# Autodesk Inventor assembly: mini sand
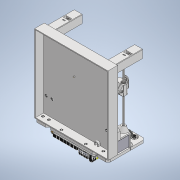
[picture p0: Inventor's stored thumbnail of the model, 180x180]
Saved by Autodesk Inventor 2022 (Build 260153000, 153)
## iProperties
Created: 2022-04-23
Part Number: mini sand
Document SubType Name: Assembly
Designer: Administrator
Title: mini sand v11
Author: Administrator
## Documents named in this file (29)
- Y:\Projects\Mini_Sand_Table\Mini Sand Table.iam
- Y:\Projects\Mini_Sand_Table\4mm x 140mm Rod.ipt
- Y:\Projects\Mini_Sand_Table\603ZZ Roller Bearing.ipt
- Y:\Projects\Mini_Sand_Table\4mm x 130mm Rod.ipt
- Y:\Projects\Mini_Sand_Table\GT2 16T Pulley.ipt
- Y:\Projects\Mini_Sand_Table\magnet.ipt
- Y:\Projects\Mini_Sand_Table\LM4UU.ipt
- Y:\Projects\Mini_Sand_Table\Table Top.ipt
- Y:\Projects\Mini_Sand_Table\NEMA 11.ipt
- Y:\Projects\Mini_Sand_Table\Belt Retainer.ipt
- Y:\Projects\Mini_Sand_Table\Magnet Mount Lower.ipt
- Y:\Projects\Mini_Sand_Table\XY Joiner HSI.iam
- Y:\Projects\Mini_Sand_Table\Idle Bearing Mount HSI.iam
- Y:\Projects\Mini_Sand_Table\M3 Hex Nut.ipt
- Y:\Projects\Mini_Sand_Table\Ball.ipt
- Y:\Projects\Mini_Sand_Table\SKR Mini E3 v3.0.ipt
- Y:\Projects\Mini_Sand_Table\Sand Cover.ipt
- Y:\Projects\Mini_Sand_Table\Magnet Mount HSI.iam
- Y:\Projects\Mini_Sand_Table\Motor Mount HSI.iam
- Y:\Projects\Mini_Sand_Table\Driver Board Mount HSI.iam
- Y:\Projects\Mini_Sand_Table\M3 x 4 mm SHCS.ipt
- Y:\Projects\Mini_Sand_Table\M3 x 25 mm  SHCS.ipt
- Y:\Projects\Mini_Sand_Table\M2.5 x 10 mm SHCS.ipt
- Y:\Projects\Mini_Sand_Table\M2.5 x 6 mm SHCS.ipt
- Y:\Projects\Mini_Sand_Table\M3 x 16 mm FHCS.ipt
- Y:\Projects\Mini_Sand_Table\M3 x 10 mm FHCS.ipt
- Y:\Projects\Mini_Sand_Table\DC Jack.ipt
- Y:\Projects\Mini_Sand_Table\DC Jack Nut.ipt
- Y:\Projects\Mini_Sand_Table\5mm M3 Brass Standoff.ipt
## Components (90 placed, 30 different names)
1. 5mm M3 Brass Standoff:5 — Insert:225
2. 5mm M3 Brass Standoff:4 — Insert:226
3. 5mm M3 Brass Standoff:3 — Insert:229
4. 5mm M3 Brass Standoff:2 — Insert:227
5. 5mm M3 Brass Standoff:1 — Insert:228
6. magnet:1 — Mate:31, Insert:107
7. 4mm x 140mm Rod:1 — Insert:60, Mate:46
8. 4mm x 140mm Rod:2 — Mate:9, Insert:61
9. 4mm x 130mm Rod:2 — Insert:95, Mate:43, Mate:45
10. 4mm x 130mm Rod:3 — Insert:87, Mate:42, Mate:44
11. GT2 16T Pulley:2 — Insert:68
12. gt2 pulley 16t v1:1 — Insert:65
13. Ball:1 — Mate:31, Tangent:1
14. Belt Retainer:2 — Insert:194, Insert:195
15. XY Joiner HSI:3 [sub-assembly] — Mate:44, Mate:45, Insert:202
16. Magnet Mount Lower:1 — Insert:105, Insert:106, Insert:158, Insert:159, Insert:196, Insert:197
17. Magnet Mount HSI:1 [sub-assembly] — Insert:105, Insert:106, Insert:107
18. Motor Mount HSI:1 [sub-assembly] — Insert:108, Insert:109, Insert:110, Insert:111, Insert:146, Insert:147
19. Motor Mount HSI:2 [sub-assembly] — Insert:112, Insert:113, Insert:114, Insert:148, Insert:149
20. table mount (1):1 [sub-assembly] — Insert:56, Insert:57, Insert:60, Insert:90, Insert:141, Angle:4, Insert:204
21. table mount (1):2 [sub-assembly] — Insert:58, Insert:59, Insert:61, Insert:89, Insert:140, Angle:3, Insert:205
22. XY Joiner HSI:2 [sub-assembly] — Insert:80, Insert:81, Insert:86, Angle:2, Insert:87, Insert:95, Insert:98, Insert:99, Insert:156, Angle:6, Insert:173, Insert:203
23. Belt Retainer:1 — Insert:82, Insert:83, Insert:198, Insert:199
24. Table Top:1 — Insert:56, Insert:57, Insert:58, Insert:59, Tangent:1, Mate:39, Mate:40, Mate:41, Insert:108, Insert:109, Insert:112, Insert:113, Insert:115, Insert:116, Insert:206, Insert:207, Insert:208, Insert:209, Insert:210, Insert:211, Insert:212, Insert:213, Insert:217, Insert:218, Insert:219, Insert:220, Insert:221, Insert:222, Insert:223, Insert:224
25. Driver Board Mount HSI:1 [sub-assembly] — Insert:115, Insert:116, Insert:142, Insert:143, Insert:144, Insert:145, Mate:47, Insert:200, Insert:201, Flush:1, Mate:48, Flush:2, Insert:225, Insert:226, Insert:227, Insert:228, Insert:229
26. Sand Cover:1 — Mate:39, Mate:40, Mate:41
27. DC Jack:1 — Insert:200
28. DC Jack Nut:1 — Insert:201
29. NEMA 11:1 — Insert:68, Insert:114, Mate:47
30. NEMA 11:2 — Insert:65, Insert:110, Insert:111
31. SKR Mini E3 v3.0:2 — Insert:117, Insert:118, Insert:119, Insert:120, Insert:121, Flush:1, Mate:48, Flush:2
32. LM4UU:3 — Mate:9, Insert:98
33. LM4UU:4 — Insert:99
34. LM4UU:5 — Insert:159, Mate:43
35. LM4UU:6 — Insert:158, Mate:42
36. LM4UU:7 — Mate:46
37. LM4UU:8
38. 603ZZ Roller Bearing:5 — Insert:81, Insert:82
39. 603ZZ Roller Bearing:6 — Insert:80, Insert:83
40. 603ZZ Roller Bearing:7
41. 603ZZ Roller Bearing:8
42. roller bearing:3 — Insert:90
43. roller bearing:4 — Insert:89
44. M3 Hex Nut:3 — Insert:141, Angle:4
45. M3 Hex Nut:4 — Insert:140, Angle:3
46. M3 Hex Nut:8
47. M3 Hex Nut:7
48. M3 Hex Nut:2 — Insert:86, Angle:2
49. M3 Hex Nut:6 — Insert:156, Angle:6
50. M3 x 4 mm SHCS:1 — Insert:117
51. M3 x 4 mm SHCS:2 — Insert:118
52. M3 x 4 mm SHCS:3 — Insert:119
53. M3 x 4 mm SHCS:4 — Insert:120
54. M3 x 4 mm SHCS:5 — Insert:121
55. M3 x 10 mm FHCS:25 — Insert:222
56. M3 x 10 mm FHCS:24 — Insert:224
57. M3 x 10 mm FHCS:23 — Insert:223
58. M3 x 10 mm FHCS:7 — Insert:219
59. M3 x 10 mm FHCS:8 — Insert:212
60. M3 x 10 mm FHCS:9 — Insert:221
61. M3 x 10 mm FHCS:10 — Insert:213
62. M3 x 10 mm FHCS:11 — Insert:220
63. M3 x 10 mm FHCS:12 — Insert:217
64. M3 x 10 mm FHCS:15 — Insert:218
65. M3 x 10 mm FHCS:17 — Insert:206
66. M3 x 10 mm FHCS:18 — Insert:207
67. M3 x 10 mm FHCS:19 — Insert:208
68. M3 x 10 mm FHCS:20 — Insert:209
69. M3 x 10 mm FHCS:21 — Insert:210
70. M3 x 10 mm FHCS:22 — Insert:211
71. M3 x 10 mm FHCS:6 — Insert:199
72. M3 x 10 mm FHCS:5 — Insert:198
73. M3 x 10 mm FHCS:4 — Insert:197
74. M3 x 10 mm FHCS:3 — Insert:196
75. M3 x 10 mm FHCS:2 — Insert:195
76. M3 x 10 mm FHCS:1 — Insert:194
77. M3 x 16 mm FHCS:1 — Insert:173
78. M3 x 16 mm FHCS:2 — Insert:203
79. M3 x 16 mm FHCS:3
80. M3 x 16 mm FHCS:4 — Insert:202
81. M3 x 25 mm  SHCS:1 — Insert:205
82. M3 x 25 mm  SHCS:2 — Insert:204
83. M2.5 x 10 mm SHCS:1 — Insert:143
84. M2.5 x 10 mm SHCS:2 — Insert:142
85. M2.5 x 10 mm SHCS:3 — Insert:145
86. M2.5 x 10 mm SHCS:4 — Insert:144
87. M2.5 x 6 mm SHCS:1 — Insert:146
88. M2.5 x 6 mm SHCS:2 — Insert:147
89. M2.5 x 6 mm SHCS:3 — Insert:148
90. M2.5 x 6 mm SHCS:4 — Insert:149
## Relationships (113: Insert 92, Mate 12, Angle 6, Flush 2, Tangent 1)
- Mate:9: 4mm x 140mm Rod:2 ↔ LM4UU:3
- Insert:56: table mount (1):1 ↔ Table Top:1
- Insert:57: table mount (1):1 ↔ Table Top:1
- Insert:58: table mount (1):2 ↔ Table Top:1
- Insert:59: table mount (1):2 ↔ Table Top:1
- Insert:60: 4mm x 140mm Rod:1 ↔ table mount (1):1
- Insert:61: 4mm x 140mm Rod:2 ↔ table mount (1):2
- Insert:65: gt2 pulley 16t v1:1 ↔ NEMA 11:2
- Insert:68: GT2 16T Pulley:2 ↔ NEMA 11:1
- Insert:80: XY Joiner HSI:2 ↔ 603ZZ Roller Bearing:6
- Insert:81: XY Joiner HSI:2 ↔ 603ZZ Roller Bearing:5
- Insert:82: Belt Retainer:1 ↔ 603ZZ Roller Bearing:5
- Insert:83: Belt Retainer:1 ↔ 603ZZ Roller Bearing:6
- Insert:86: XY Joiner HSI:2 ↔ M3 Hex Nut:2
- Angle:2 (0 deg): XY Joiner HSI:2 ↔ M3 Hex Nut:2
- Insert:87: 4mm x 130mm Rod:3 ↔ XY Joiner HSI:2
- Insert:89: table mount (1):2 ↔ roller bearing:4
- Insert:90: table mount (1):1 ↔ roller bearing:3
- Insert:95: 4mm x 130mm Rod:2 ↔ XY Joiner HSI:2
- Insert:98: XY Joiner HSI:2 ↔ LM4UU:3
- Insert:99: XY Joiner HSI:2 ↔ LM4UU:4
- Mate:31: magnet:1 ↔ Ball:1
- Tangent:1: Ball:1 ↔ Table Top:1
- Mate:39: Table Top:1 ↔ Sand Cover:1
- Mate:40: Table Top:1 ↔ Sand Cover:1
- Mate:41: Table Top:1 ↔ Sand Cover:1
- Insert:105: Magnet Mount Lower:1 ↔ Magnet Mount HSI:1
- Insert:106: Magnet Mount Lower:1 ↔ Magnet Mount HSI:1
- Insert:107: magnet:1 ↔ Magnet Mount HSI:1
- Insert:108: Motor Mount HSI:1 ↔ Table Top:1
- Insert:109: Motor Mount HSI:1 ↔ Table Top:1
- Insert:110: Motor Mount HSI:1 ↔ NEMA 11:2
- Insert:111: Motor Mount HSI:1 ↔ NEMA 11:2
- Insert:112: Motor Mount HSI:2 ↔ Table Top:1
- Insert:113: Motor Mount HSI:2 ↔ Table Top:1
- Insert:114: Motor Mount HSI:2 ↔ NEMA 11:1
- Insert:115: Table Top:1 ↔ Driver Board Mount HSI:1
- Insert:116: Table Top:1 ↔ Driver Board Mount HSI:1
- Insert:117: SKR Mini E3 v3.0:2 ↔ M3 x 4 mm SHCS:1
- Insert:118: SKR Mini E3 v3.0:2 ↔ M3 x 4 mm SHCS:2
- Insert:119: SKR Mini E3 v3.0:2 ↔ M3 x 4 mm SHCS:3
- Insert:120: SKR Mini E3 v3.0:2 ↔ M3 x 4 mm SHCS:4
- Insert:121: SKR Mini E3 v3.0:2 ↔ M3 x 4 mm SHCS:5
- Insert:140: table mount (1):2 ↔ M3 Hex Nut:4
- Angle:3 (0 deg): table mount (1):2 ↔ M3 Hex Nut:4
- Insert:141: table mount (1):1 ↔ M3 Hex Nut:3
- Angle:4 (0 deg): table mount (1):1 ↔ M3 Hex Nut:3
- Insert:142: Driver Board Mount HSI:1 ↔ M2.5 x 10 mm SHCS:2
- Insert:143: Driver Board Mount HSI:1 ↔ M2.5 x 10 mm SHCS:1
- Insert:144: Driver Board Mount HSI:1 ↔ M2.5 x 10 mm SHCS:4
- Insert:145: Driver Board Mount HSI:1 ↔ M2.5 x 10 mm SHCS:3
- Insert:146: Motor Mount HSI:1 ↔ M2.5 x 6 mm SHCS:1
- Insert:147: Motor Mount HSI:1 ↔ M2.5 x 6 mm SHCS:2
- Insert:148: Motor Mount HSI:2 ↔ M2.5 x 6 mm SHCS:3
- Insert:149: Motor Mount HSI:2 ↔ M2.5 x 6 mm SHCS:4
- Insert:156: XY Joiner HSI:2 ↔ M3 Hex Nut:6
- Angle:6 (0 deg): XY Joiner HSI:2 ↔ M3 Hex Nut:6
- Insert:158: Magnet Mount Lower:1 ↔ LM4UU:6
- Insert:159: Magnet Mount Lower:1 ↔ LM4UU:5
- Mate:42: 4mm x 130mm Rod:3 ↔ LM4UU:6
- Mate:43: 4mm x 130mm Rod:2 ↔ LM4UU:5
- Insert:173: XY Joiner HSI:2 ↔ M3 x 16 mm FHCS:1
- [Insert]: XY Joiner HSI:3 ↔ 603ZZ Roller Bearing:8
- [Insert]: XY Joiner HSI:3 ↔ 603ZZ Roller Bearing:7
- [Insert]: Belt Retainer:2 ↔ 603ZZ Roller Bearing:7
- [Insert]: Belt Retainer:2 ↔ 603ZZ Roller Bearing:8
- [Insert]: XY Joiner HSI:3 ↔ M3 Hex Nut:7
- [Angle] (0 deg): XY Joiner HSI:3 ↔ M3 Hex Nut:7
- [Insert]: XY Joiner HSI:3 ↔ LM4UU:7
- [Insert]: XY Joiner HSI:3 ↔ LM4UU:8
- [Insert]: XY Joiner HSI:3 ↔ M3 Hex Nut:8
- [Angle] (0 deg): XY Joiner HSI:3 ↔ M3 Hex Nut:8
- [Insert]: XY Joiner HSI:3 ↔ M3 x 16 mm FHCS:3
- Mate:44: 4mm x 130mm Rod:3 ↔ XY Joiner HSI:3
- Mate:45: 4mm x 130mm Rod:2 ↔ XY Joiner HSI:3
- Mate:46: 4mm x 140mm Rod:1 ↔ LM4UU:7
- Mate:47: Driver Board Mount HSI:1 ↔ NEMA 11:1
- Insert:194: Belt Retainer:2 ↔ M3 x 10 mm FHCS:1
- Insert:195: Belt Retainer:2 ↔ M3 x 10 mm FHCS:2
- Insert:196: Magnet Mount Lower:1 ↔ M3 x 10 mm FHCS:3
- Insert:197: Magnet Mount Lower:1 ↔ M3 x 10 mm FHCS:4
- Insert:198: Belt Retainer:1 ↔ M3 x 10 mm FHCS:5
- Insert:199: Belt Retainer:1 ↔ M3 x 10 mm FHCS:6
- Insert:200: Driver Board Mount HSI:1 ↔ DC Jack:1
- Insert:201: Driver Board Mount HSI:1 ↔ DC Jack Nut:1
- Insert:202: XY Joiner HSI:3 ↔ M3 x 16 mm FHCS:4
- Insert:203: XY Joiner HSI:2 ↔ M3 x 16 mm FHCS:2
- Insert:204: table mount (1):1 ↔ M3 x 25 mm  SHCS:2
- Insert:205: table mount (1):2 ↔ M3 x 25 mm  SHCS:1
- Insert:206: Table Top:1 ↔ M3 x 10 mm FHCS:17
- Insert:207: Table Top:1 ↔ M3 x 10 mm FHCS:18
- Insert:208: Table Top:1 ↔ M3 x 10 mm FHCS:19
- Insert:209: Table Top:1 ↔ M3 x 10 mm FHCS:20
- Insert:210: Table Top:1 ↔ M3 x 10 mm FHCS:21
- Insert:211: Table Top:1 ↔ M3 x 10 mm FHCS:22
- Insert:212: Table Top:1 ↔ M3 x 10 mm FHCS:8
- Insert:213: Table Top:1 ↔ M3 x 10 mm FHCS:10
- Insert:217: Table Top:1 ↔ M3 x 10 mm FHCS:12
- Insert:218: Table Top:1 ↔ M3 x 10 mm FHCS:15
- Insert:219: Table Top:1 ↔ M3 x 10 mm FHCS:7
- Insert:220: Table Top:1 ↔ M3 x 10 mm FHCS:11
- Insert:221: Table Top:1 ↔ M3 x 10 mm FHCS:9
- Flush:1 (2 mm): Driver Board Mount HSI:1 ↔ SKR Mini E3 v3.0:2
- Mate:48 (5 mm): Driver Board Mount HSI:1 ↔ SKR Mini E3 v3.0:2
- Flush:2 (3.35 mm): Driver Board Mount HSI:1 ↔ SKR Mini E3 v3.0:2
- Insert:222: Table Top:1 ↔ M3 x 10 mm FHCS:25
- Insert:223: Table Top:1 ↔ M3 x 10 mm FHCS:23
- Insert:224: Table Top:1 ↔ M3 x 10 mm FHCS:24
- Insert:225: 5mm M3 Brass Standoff:5 ↔ Driver Board Mount HSI:1
- Insert:226: 5mm M3 Brass Standoff:4 ↔ Driver Board Mount HSI:1
- Insert:227: 5mm M3 Brass Standoff:2 ↔ Driver Board Mount HSI:1
- Insert:228: 5mm M3 Brass Standoff:1 ↔ Driver Board Mount HSI:1
- Insert:229: 5mm M3 Brass Standoff:3 ↔ Driver Board Mount HSI:1
## Named parameters: d263_d240 = 0 mm, d264_d241 = 0 deg, d265_d159 = 0 mm, d266_d160 = 0 mm, d267_d131 = 0 mm, d268_d132 = 0 mm, d269_d133 = 0 mm, d270_d134 = 0 mm, d271_d137 = 0 mm, d272_d138 = 0 deg, d275_d261 = 0 mm
